# Autodesk Inventor assembly: leg_1_MIR
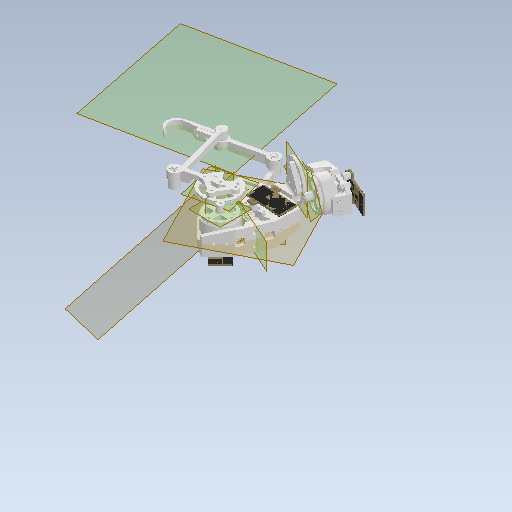
[picture p0: Inventor's stored thumbnail of the model, 512x512]
Saved by Autodesk Inventor 2023 (Build 270158000, 158)
## iProperties
Created: 2020-12-08
Part Number: leg_1_MIR
Document SubType Name: Assembly
Designer: Shuang Peng
Author: Shuang Peng
## Documents named in this file (12)
- D:\projects-3\biped_tiny\hardware\leg_1_MIR.iam
- D:\projects-3\biped_tiny\hardware\reducer_1_MIR.iam
- D:\projects-3\biped_tiny\hardware\leg_holder_2_MIR.ipt
- D:\projects-3\biped_tiny\hardware\leg_link_1_MIR.ipt
- D:\projects-3\biped_tiny\hardware\leg_link_2_MIR.ipt
- D:\projects-3\biped_tiny\hardware\leg_link_4_MIR.ipt
- D:\projects-3\biped_tiny\hardware\leg_link_3_m_MIR.ipt
- D:\projects-3\biped_tiny\hardware\foot_2_MIR.ipt
- D:\projects-3\biped_tiny\hardware\bearing_3_6_2_MIR.ipt
- D:\projects-3\biped_tiny\hardware\pin_3_15_MIR.ipt
- D:\projects-3\biped_tiny\hardware\wh_ass_3_MIR.iam
- D:\projects-3\biped_tiny\hardware\body_conn_1_MIR.ipt
## Components (22 placed, 11 different names)
1. reducer_1_MIR:1 [sub-assembly] — Tangent:1, Flush:1, Mate:4, Insert:2, Insert:1, Symmetry:1, Insert:29
2. reducer_1_MIR:2 [sub-assembly] — Tangent:1, Flush:1, Mate:3, Insert:4, Insert:3, Flush:4, Symmetry:1, Insert:30
3. leg_holder_2_MIR:1 — Insert:4, Insert:3, Insert:2, Insert:1, Flush:4, Insert:28, Insert:29, Angle:1
4. leg_link_1_MIR:1 — Flush:5, Insert:9, Flush:6, Insert:16, Insert:19, Insert:18, Flush:7, Insert:23, Insert:22, Insert:25, Insert:24
5. leg_link_2_MIR:1 — Insert:9, Flush:6, Insert:26, Insert:34, Insert:33
6. leg_link_4_MIR:1 — Insert:17, Insert:20, Insert:21, Insert:32, Insert:31
7. leg_link_3_m_MIR:1 — Insert:17, Insert:16, Insert:27, Insert:28
8. foot_2_MIR:1 — Insert:19, Insert:18, Flush:7
9. bearing_3_6_2_MIR:1 — Insert:20
10. bearing_3_6_2_MIR:2 — Insert:21
11. bearing_3_6_2_MIR:3 — Insert:23
12. bearing_3_6_2_MIR:4 — Insert:22
13. bearing_3_6_2_MIR:5 — Insert:25
14. bearing_3_6_2_MIR:6 — Insert:24
15. pin_3_15_MIR:1 — Insert:26
16. pin_3_15_MIR:2 — Insert:27
17. pin_3_15_MIR:3 — Insert:28
18. reducer_1_MIR:3 [sub-assembly] — Insert:35, Angle:1
19. wh_ass_3_MIR:1 [sub-assembly] — Insert:34, Insert:33, Insert:30
20. wh_ass_3_MIR:2 [sub-assembly] — Insert:32, Insert:31, Insert:29
21. wh_ass_3_MIR:3 [sub-assembly] — Insert:35, Insert:39, Insert:38
22. body_conn_1_MIR:1 — Insert:39, Insert:38, Insert:28, Insert:29
## Relationships (39: Insert 29, Mate 6, Tangent 1, Flush 1, Symmetry 1, Angle 1)
- Tangent:1 (2 mm): reducer_1_MIR:1 ↔ reducer_1_MIR:2
- Flush:1 (-9.5 mm): reducer_1_MIR:1 ↔ reducer_1_MIR:2
- Mate:4: reducer_1_MIR:1
- Mate:3: reducer_1_MIR:2
- Insert:4: reducer_1_MIR:2 ↔ leg_holder_2_MIR:1
- Insert:3: reducer_1_MIR:2 ↔ leg_holder_2_MIR:1
- Insert:2: reducer_1_MIR:1 ↔ leg_holder_2_MIR:1
- Insert:1: reducer_1_MIR:1 ↔ leg_holder_2_MIR:1
- Flush:4 [Mate]: reducer_1_MIR:2 ↔ leg_holder_2_MIR:1
- Symmetry:1: reducer_1_MIR:1 ↔ reducer_1_MIR:2
- Flush:5 [Mate]: leg_link_1_MIR:1
- Insert:9: leg_link_1_MIR:1 ↔ leg_link_2_MIR:1
- Flush:6 [Mate]: leg_link_1_MIR:1 ↔ leg_link_2_MIR:1
- Insert:17: leg_link_4_MIR:1 ↔ leg_link_3_m_MIR:1
- Insert:16: leg_link_1_MIR:1 ↔ leg_link_3_m_MIR:1
- Insert:19: leg_link_1_MIR:1 ↔ foot_2_MIR:1
- Insert:18: leg_link_1_MIR:1 ↔ foot_2_MIR:1
- Flush:7 [Mate]: leg_link_1_MIR:1 ↔ foot_2_MIR:1
- Insert:20: leg_link_4_MIR:1 ↔ bearing_3_6_2_MIR:1
- Insert:21: leg_link_4_MIR:1 ↔ bearing_3_6_2_MIR:2
- Insert:23: leg_link_1_MIR:1 ↔ bearing_3_6_2_MIR:3
- Insert:22: leg_link_1_MIR:1 ↔ bearing_3_6_2_MIR:4
- Insert:25: leg_link_1_MIR:1 ↔ bearing_3_6_2_MIR:5
- Insert:24: leg_link_1_MIR:1 ↔ bearing_3_6_2_MIR:6
- Insert:26: leg_link_2_MIR:1 ↔ pin_3_15_MIR:1
- Insert:27: leg_link_3_m_MIR:1 ↔ pin_3_15_MIR:2
- Insert:28: leg_link_3_m_MIR:1 ↔ pin_3_15_MIR:3
- Insert:34: leg_link_2_MIR:1 ↔ wh_ass_3_MIR:1
- Insert:33: leg_link_2_MIR:1 ↔ wh_ass_3_MIR:1
- Insert:30: reducer_1_MIR:2 ↔ wh_ass_3_MIR:1
- Insert:32: leg_link_4_MIR:1 ↔ wh_ass_3_MIR:2
- Insert:31: leg_link_4_MIR:1 ↔ wh_ass_3_MIR:2
- Insert:29: reducer_1_MIR:1 ↔ wh_ass_3_MIR:2
- Insert:35: reducer_1_MIR:3 ↔ wh_ass_3_MIR:3
- Insert:39: wh_ass_3_MIR:3 ↔ body_conn_1_MIR:1
- Insert:38: wh_ass_3_MIR:3 ↔ body_conn_1_MIR:1
- Insert:28: leg_holder_2_MIR:1 ↔ body_conn_1_MIR:1
- Insert:29: leg_holder_2_MIR:1 ↔ body_conn_1_MIR:1
- Angle:1 (0 deg): leg_holder_2_MIR:1 ↔ reducer_1_MIR:3
